# Autodesk Inventor assembly: X-axis Driver Holder assy
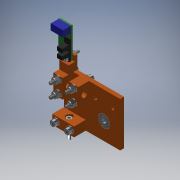
[picture p0: Inventor's stored thumbnail of the model, 180x180]
Saved by Autodesk Inventor 2018 (Build 220112000, 112)
## iProperties
Created: 2017-10-03
Part Number: X-axis Driver Holder assy
Document SubType Name: Assembly
Designer: Gabriel Smolnycki
Author: Gabriel Smolnycki
## Documents named in this file (14)
- H:\dev\planb\mechanics\V1INV\Subassemblies\X-axis Driver Holder assy.iam
- H:\dev\planb\mechanics\V1INV\X-axis\X-axis Driver Holder.ipt
- H:\dev\planb\mechanics\V1INV\Hardware\5x16 SS Ball Bearing (6153K150).ipt
- H:\dev\planb\mechanics\V1INV\Electronics\Endstop.ipt
- H:\dev\planb\mechanics\V1INV\Hardware\M3x16 SS SHCS.ipt
- H:\dev\planb\mechanics\V1INV\Hardware\M3 SS Washer.ipt
- H:\dev\planb\mechanics\V1INV\Hardware\M3 SS Nut.ipt
- H:\dev\planb\mechanics\V1INV\X-axis\X-axis Rod Holder.ipt
- H:\dev\planb\mechanics\V1INV\Hardware\M4x30 SS SHCS.ipt
- H:\dev\planb\mechanics\V1INV\Hardware\M4 SS Washer.ipt
- H:\dev\planb\mechanics\V1INV\Hardware\M4 SS Locknut.ipt
- H:\dev\planb\mechanics\V1INV\X-axis\X-axis Holder Coupler.ipt
- H:\dev\planb\mechanics\V1INV\Hardware\M4x20 SS SHCS.ipt
- H:\dev\planb\mechanics\V1INV\Hardware\M4x40 SS SHCS.ipt
## Components (36 placed, 13 different names)
1. X-axis Driver Holder:1 — Insert:1, Insert:2, Mate:1, Insert:4, Insert:6, Insert:7, Insert:8, Insert:9, Insert:10, Insert:11, Insert:12, Insert:13, Insert:28, Insert:29, Insert:32, Insert:33
2. 5x16 SS Ball Bearing (6153K150):1 — Insert:1
3. Endstop:1 — Insert:2, Mate:1, Insert:3
4. M3x16 SS SHCS:1 — Insert:3
5. M3 SS Washer:1 — Insert:4, Insert:5
6. M3 SS Nut:1 — Insert:5
7. X-axis Rod Holder:1 — Insert:6, Insert:7, Insert:14, Insert:15
8. X-axis Rod Holder:2 — Insert:8, Insert:9, Insert:16, Insert:17
9. M4x30 SS SHCS:1 — Insert:21
10. M4x30 SS SHCS:2 — Insert:20
11. M4x30 SS SHCS:3 — Insert:19
12. M4x30 SS SHCS:4 — Insert:18
13. M4 SS Washer:1 — Insert:13, Insert:20
14. M4 SS Washer:2 — Insert:10, Insert:21
15. M4 SS Washer:3 — Insert:12, Insert:19
16. M4 SS Washer:4 — Insert:11, Insert:18
17. M4 SS Washer:5 — Insert:17, Insert:23
18. M4 SS Washer:6 — Insert:16, Insert:22
19. M4 SS Washer:7 — Insert:15, Insert:25
20. M4 SS Washer:8 — Insert:14, Insert:24
21. M4 SS Locknut:1 — Insert:25
22. M4 SS Locknut:2 — Insert:24
23. M4 SS Locknut:3 — Insert:23
24. M4 SS Locknut:4 — Insert:22
25. X-axis Holder Coupler:1 — Insert:30, Insert:32, Insert:33, Insert:34, Insert:35
26. X-axis Holder Coupler:2 — Insert:28, Insert:29, Insert:31, Insert:36, Insert:37
27. M4x20 SS SHCS:1 — Insert:30
28. M4x20 SS SHCS:2 — Insert:31
29. M4x40 SS SHCS:1 — Insert:41
30. M4x40 SS SHCS:2 — Insert:40
31. M4 SS Washer:9 — Insert:35, Insert:41
32. M4 SS Washer:10 — Insert:34, Insert:40
33. M4 SS Washer:11 — Insert:36, Insert:39
34. M4 SS Washer:12 — Insert:37, Insert:38
35. M4 SS Locknut:5 — Insert:39
36. M4 SS Locknut:6 — Insert:38
## Relationships (40: Insert 39, Mate 1)
- Insert:1: X-axis Driver Holder:1 ↔ 5x16 SS Ball Bearing (6153K150):1
- Insert:2: X-axis Driver Holder:1 ↔ Endstop:1
- Mate:1: X-axis Driver Holder:1 ↔ Endstop:1
- Insert:3: Endstop:1 ↔ M3x16 SS SHCS:1
- Insert:4: X-axis Driver Holder:1 ↔ M3 SS Washer:1
- Insert:5: M3 SS Washer:1 ↔ M3 SS Nut:1
- Insert:6: X-axis Driver Holder:1 ↔ X-axis Rod Holder:1
- Insert:7: X-axis Driver Holder:1 ↔ X-axis Rod Holder:1
- Insert:8: X-axis Driver Holder:1 ↔ X-axis Rod Holder:2
- Insert:9: X-axis Driver Holder:1 ↔ X-axis Rod Holder:2
- Insert:10: X-axis Driver Holder:1 ↔ M4 SS Washer:2
- Insert:11: X-axis Driver Holder:1 ↔ M4 SS Washer:4
- Insert:12: X-axis Driver Holder:1 ↔ M4 SS Washer:3
- Insert:13: X-axis Driver Holder:1 ↔ M4 SS Washer:1
- Insert:14: X-axis Rod Holder:1 ↔ M4 SS Washer:8
- Insert:15: X-axis Rod Holder:1 ↔ M4 SS Washer:7
- Insert:16: X-axis Rod Holder:2 ↔ M4 SS Washer:6
- Insert:17: X-axis Rod Holder:2 ↔ M4 SS Washer:5
- Insert:18: M4x30 SS SHCS:4 ↔ M4 SS Washer:4
- Insert:19: M4x30 SS SHCS:3 ↔ M4 SS Washer:3
- Insert:20: M4x30 SS SHCS:2 ↔ M4 SS Washer:1
- Insert:21: M4x30 SS SHCS:1 ↔ M4 SS Washer:2
- Insert:22: M4 SS Washer:6 ↔ M4 SS Locknut:4
- Insert:23: M4 SS Washer:5 ↔ M4 SS Locknut:3
- Insert:24: M4 SS Washer:8 ↔ M4 SS Locknut:2
- Insert:25: M4 SS Washer:7 ↔ M4 SS Locknut:1
- Insert:28: X-axis Driver Holder:1 ↔ X-axis Holder Coupler:2
- Insert:29: X-axis Driver Holder:1 ↔ X-axis Holder Coupler:2
- Insert:30: X-axis Holder Coupler:1 ↔ M4x20 SS SHCS:1
- Insert:31: X-axis Holder Coupler:2 ↔ M4x20 SS SHCS:2
- Insert:32: X-axis Driver Holder:1 ↔ X-axis Holder Coupler:1
- Insert:33: X-axis Driver Holder:1 ↔ X-axis Holder Coupler:1
- Insert:34: X-axis Holder Coupler:1 ↔ M4 SS Washer:10
- Insert:35: X-axis Holder Coupler:1 ↔ M4 SS Washer:9
- Insert:36: X-axis Holder Coupler:2 ↔ M4 SS Washer:11
- Insert:37: X-axis Holder Coupler:2 ↔ M4 SS Washer:12
- Insert:38: M4 SS Washer:12 ↔ M4 SS Locknut:6
- Insert:39: M4 SS Washer:11 ↔ M4 SS Locknut:5
- Insert:40: M4x40 SS SHCS:2 ↔ M4 SS Washer:10
- Insert:41: M4x40 SS SHCS:1 ↔ M4 SS Washer:9
